# Autodesk Inventor assembly: stepCounterHousing
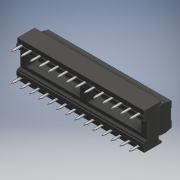
[picture p0: Inventor's stored thumbnail of the model, 180x180]
Saved by Autodesk Inventor 2018 (Build 220112000, 112)
## iProperties
Created: 2017-04-13
Part Number: stepCounterHousing
Document SubType Name: Assembly
Designer: kampe_000
Author: kampe_000
## Documents named in this file (3)
- D:\Kod\stepCounter\CAD\Inventor Project\stepCounterHousing.iam
- D:\Kod\stepCounter\CAD\Inventor Project\assembly\atmega.iam
- D:\Kod\stepCounter\CAD\Inventor Project\assembly\socket.iam
## Components (2 placed, 2 different names)
1. atmega:1 [sub-assembly] — Mate:1, Flush:1, Mate:2
2. socket:1 [sub-assembly] — Mate:1, Flush:1, Mate:2, Flush:2
## Relationships (4: Mate 2, Flush 2)
- Mate:1: atmega:1 ↔ socket:1
- Flush:1: atmega:1 ↔ socket:1
- Mate:2 (0.1 mm): atmega:1 ↔ socket:1
- Flush:2: socket:1
